# Autodesk Inventor assembly: tool
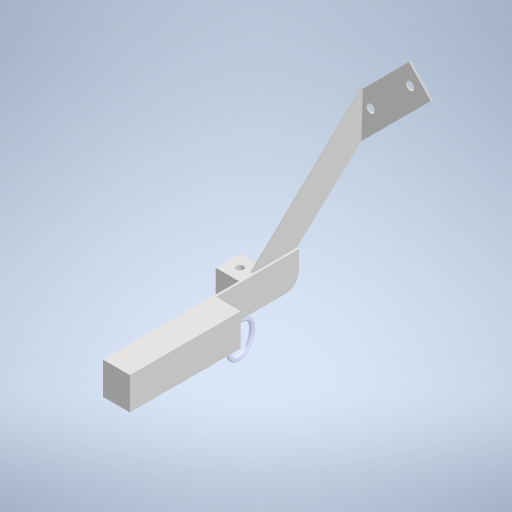
[picture p0: Inventor's stored thumbnail of the model, 512x512]
Saved by Autodesk Inventor 2023 (Build 270158000, 158)
## iProperties
Created: 2023-06-08
Part Number: tool
Document SubType Name: Weldment
Designer: robin
Weld Material: Welded Aluminum-6061
Author: robin
## Documents named in this file (4)
- C:\Users\robin\Desktop\probotica 2023-1\tool.iam
- C:\Users\robin\Desktop\probotica 2023-1\ventosas.ipt
- C:\Users\robin\Desktop\probotica 2023-1\Gancho.ipt
- C:\Users\robin\Desktop\probotica 2023-1\adaptador.ipt
## Components (3 placed, 3 different names)
1. ventosas:1 — Mate:3, Flush:1
2. Gancho:1 — Cylindrical:1, Mate:2
3. adaptador:1 — Cylindrical:1, Mate:2, Mate:3, Flush:1
## Relationships (4: Mate 2, CylindricalJoint 1, Flush 1)
- Cylindrical:1: Gancho:1 ↔ adaptador:1
- Mate:2: Gancho:1 ↔ adaptador:1
- Mate:3: ventosas:1 ↔ adaptador:1
- Flush:1: ventosas:1 ↔ adaptador:1
